# Autodesk Inventor assembly: Bed
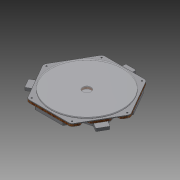
[picture p0: Inventor's stored thumbnail of the model, 180x180]
Saved by Autodesk Inventor 2014 (Build 180170000, 170)
## iProperties
Created: 2014-11-15
Part Number: Bed
Document SubType Name: Assembly
Designer: ThatOtherGuy
Author: ThatOtherGuy
## Documents named in this file (5)
- U:\Hobbies\Inventor\KosselCNC1515\Frame\Bed.iam
- U:\Hobbies\Inventor\KosselCNC1515\Build_170mm_Borosilicate.ipt
- U:\Hobbies\Inventor\KosselCNC1515\Frame\Frame_Bed.ipt
- U:\Hobbies\Inventor\KosselCNC1515\Frame\Heatbed_170mm_Hex.ipt
- U:\Hobbies\Inventor\KosselCNC1515\Frame\Heatbed_Insulator_Cork.ipt
## Components (4 placed, 4 different names)
1. Build_170mm_Borosilicate:1 — Mate:1, Mate:2
2. Frame_Bed:1 — Mate:3, Flush:1, Flush:2
3. Heatbed_170mm_Hex:1 — Mate:1, Mate:2, Flush:3, Mate:5, Flush:4
4. Heatbed_Insulator_Cork:1 — Mate:3, Flush:1, Flush:2, Flush:3, Mate:5, Flush:4
## Relationships (8: Mate 4, Flush 4)
- Mate:1: Build_170mm_Borosilicate:1 ↔ Heatbed_170mm_Hex:1
- Mate:2: Build_170mm_Borosilicate:1 ↔ Heatbed_170mm_Hex:1
- Mate:3: Frame_Bed:1 ↔ Heatbed_Insulator_Cork:1
- Flush:1: Frame_Bed:1 ↔ Heatbed_Insulator_Cork:1
- Flush:2: Frame_Bed:1 ↔ Heatbed_Insulator_Cork:1
- Flush:3: Heatbed_170mm_Hex:1 ↔ Heatbed_Insulator_Cork:1
- Mate:5: Heatbed_170mm_Hex:1 ↔ Heatbed_Insulator_Cork:1
- Flush:4: Heatbed_170mm_Hex:1 ↔ Heatbed_Insulator_Cork:1
